# Autodesk Inventor assembly: EX_ONE
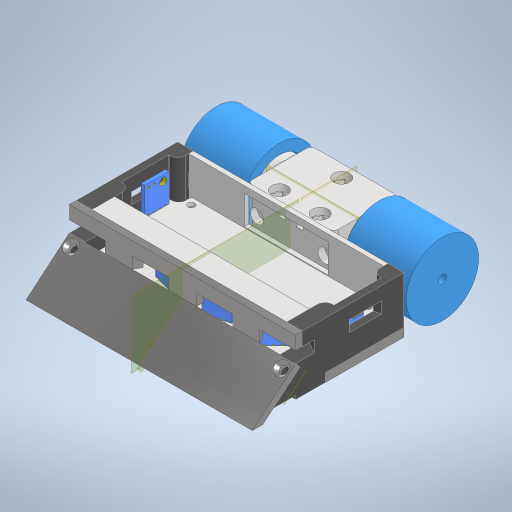
[picture p0: Inventor's stored thumbnail of the model, 512x512]
Saved by Autodesk Inventor 2023 (Build 270158000, 158)
## iProperties
Created: 2025-01-11
Part Number: EX_ONE
Document SubType Name: Assembly
Designer: kamil
Author: kamil
## Documents named in this file (15)
- C:\Users\kamil\Documents\PROJECTS - repos\EX_ONE_minisumo\mechanics\inventor_parts\EX_ONE.iam
- C:\Users\kamil\Documents\PROJECTS - repos\EX_ONE_minisumo\mechanics\inventor_parts\faulhaber_motor.ipt
- C:\Users\kamil\Documents\PROJECTS - repos\EX_ONE_minisumo\mechanics\inventor_parts\motors_mount.ipt
- C:\Users\kamil\Documents\PROJECTS - repos\EX_ONE_minisumo\mechanics\inventor_parts\kolo_tetsowe.ipt
- C:\Users\kamil\Documents\PROJECTS - repos\EX_ONE_minisumo\mechanics\inventor_parts\podstawa.ipt
- C:\Users\kamil\Documents\PROJECTS - repos\EX_ONE_minisumo\mechanics\inventor_parts\nóź.ipt
- C:\Users\kamil\Documents\PROJECTS - repos\EX_ONE_minisumo\mechanics\inventor_parts\TOF_VL53L0X (1).ipt
- C:\Users\kamil\Documents\PROJECTS - repos\EX_ONE_minisumo\mechanics\inventor_parts\pcb_pre.ipt
- C:\Users\kamil\Documents\PROJECTS - repos\EX_ONE_minisumo\mechanics\inventor_parts\minisunmo_testowe.ipt
- C:\Users\kamil\Documents\PROJECTS - repos\EX_ONE_minisumo\mechanics\inventor_parts\ściana.ipt
- C:\Users\kamil\Documents\PROJECTS - repos\EX_ONE_minisumo\mechanics\inventor_parts\ściana_MIR.ipt
- C:\Users\kamil\Documents\PROJECTS - repos\EX_ONE_minisumo\mechanics\inventor_parts\przod.ipt
- C:\Users\kamil\Documents\PROJECTS - repos\EX_ONE_minisumo\mechanics\inventor_parts\oslona.ipt
- C:\Users\kamil\Documents\PROJECTS - repos\EX_ONE_minisumo\mechanics\inventor_parts\pokrywa.ipt
- C:\Users\kamil\Documents\PROJECTS - repos\EX_ONE_minisumo\mechanics\inventor_parts\belka.ipt
## Components (21 placed, 14 different names)
1. faulhaber_motor:1 — Równoległe:31, Zestawiające:31
2. faulhaber_motor:2 — Równoległe:32, Zestawiające:30
3. motors_mount:1 — Zestawiające:9, Równoległe:23, Zestawiające:29, Równoległe:31, Równoległe:32, Zestawiające:30, Zestawiające:31, Zestawiające:32, Zestawiające:33
4. kolo_tetsowe:1 — Zestawiające:33, Równoległe:33
5. nóź:1
6. kolo_tetsowe:2 — Zestawiające:9, Zestawiające:32, Równoległe:34
7. pcb_pre:1 — Zestawiające:11, Równoległe:18
8. TOF_VL53L0X (1):1 — Zestawiające:11, Równoległe:10, Równoległe:11, Równoległe:15, Równoległe:18
9. TOF_VL53L0X (1):2 — Równoległe:11, Równoległe:15
10. TOF_VL53L0X (1):3 — Równoległe:10, Równoległe:14, Kątowe:5, Równoległe:24, Zestawiające:21, Zestawiające:23, Równoległe:26, Kątowe:8
11. TOF_VL53L0X (1):5 — Równoległe:25, Zestawiające:24, Kątowe:7, Zestawiające:26
12. TOF_VL53L0X (1):6 — Równoległe:14, Kątowe:5, Równoległe:26, Zestawiające:25, Kątowe:8, Zestawiające:27
13. minisunmo_testowe:1
14. ściana:1 — Zestawiające:18, Równoległe:21, Zestawiające:19, Równoległe:22, Symetria:1, Zestawiające:28, Równoległe:27, Równoległe:28, Równoległe:29, Równoległe:30, Równoległe:33
15. ściana_MIR:1 — Symetria:1, Równoległe:34
16. przod:1 — Zestawiające:18, Równoległe:21, Zestawiające:19, Kątowe:6, Zestawiające:22, Zestawiające:23, Zestawiające:26, Zestawiające:27
17. oslona:1 — Równoległe:22
18. pokrywa:1 — Równoległe:23
19. TOF_VL53L0X (1):7 — Kątowe:6, Równoległe:24, Zestawiające:20, Zestawiające:22, Równoległe:25, Kątowe:7
20. belka:1 — Zestawiające:28, Równoległe:27, Równoległe:28
21. podstawa:1 — Zestawiające:29, Równoległe:29, Równoległe:30
## Relationships (42: Flush 19, Mate 18, Angle 4, Symmetry 1)
- Zestawiające:9 [Mate]: motors_mount:1 ↔ kolo_tetsowe:2
- Zestawiające:11 [Mate]: pcb_pre:1 ↔ TOF_VL53L0X (1):1
- Równoległe:10 [Flush]: TOF_VL53L0X (1):1 ↔ TOF_VL53L0X (1):3
- Równoległe:11 [Flush]: TOF_VL53L0X (1):1 ↔ TOF_VL53L0X (1):2
- Równoległe:14 [Flush]: TOF_VL53L0X (1):3 ↔ TOF_VL53L0X (1):6
- Równoległe:15 [Flush]: TOF_VL53L0X (1):1 ↔ TOF_VL53L0X (1):2
- Kątowe:5 [Angle] (30 deg): TOF_VL53L0X (1):3 ↔ TOF_VL53L0X (1):6
- Równoległe:18 [Flush] (2 mm): pcb_pre:1 ↔ TOF_VL53L0X (1):1
- Zestawiające:18 [Mate]: ściana:1 ↔ przod:1
- Równoległe:21 [Flush]: ściana:1 ↔ przod:1
- Zestawiające:19 [Mate]: ściana:1 ↔ przod:1
- Równoległe:22 [Flush]: ściana:1 ↔ oslona:1
- Równoległe:23 [Flush]: motors_mount:1 ↔ pokrywa:1
- Kątowe:6 [Angle] (-195 deg): przod:1 ↔ TOF_VL53L0X (1):7
- Równoległe:24 [Flush]: TOF_VL53L0X (1):3 ↔ TOF_VL53L0X (1):7
- Symetria:1 [Symmetry]: ściana:1 ↔ ściana_MIR:1
- Zestawiające:20 [Mate] (10 mm): TOF_VL53L0X (1):7
- Zestawiające:21 [Mate] (-10 mm): TOF_VL53L0X (1):3
- Zestawiające:22 [Mate] (2 mm): przod:1 ↔ TOF_VL53L0X (1):7
- Zestawiające:23 [Mate] (2 mm): TOF_VL53L0X (1):3 ↔ przod:1
- Równoległe:25 [Flush]: TOF_VL53L0X (1):5 ↔ TOF_VL53L0X (1):7
- Równoległe:26 [Flush]: TOF_VL53L0X (1):3 ↔ TOF_VL53L0X (1):6
- Zestawiające:24 [Mate] (34 mm): TOF_VL53L0X (1):5
- Zestawiające:25 [Mate] (-34 mm): TOF_VL53L0X (1):6
- Kątowe:7 [Angle] (30 deg): TOF_VL53L0X (1):5 ↔ TOF_VL53L0X (1):7
- Kątowe:8 [Angle] (30 deg): TOF_VL53L0X (1):3 ↔ TOF_VL53L0X (1):6
- Zestawiające:26 [Mate] (5 mm): TOF_VL53L0X (1):5 ↔ przod:1
- Zestawiające:27 [Mate] (5 mm): TOF_VL53L0X (1):6 ↔ przod:1
- Zestawiające:28 [Mate]: ściana:1 ↔ belka:1
- Równoległe:27 [Flush]: ściana:1 ↔ belka:1
- Równoległe:28 [Flush]: ściana:1 ↔ belka:1
- Zestawiające:29 [Mate]: motors_mount:1 ↔ podstawa:1
- Równoległe:29 [Flush]: ściana:1 ↔ podstawa:1
- Równoległe:30 [Flush]: ściana:1 ↔ podstawa:1
- Równoległe:31 [Flush]: faulhaber_motor:1 ↔ motors_mount:1
- Równoległe:32 [Flush]: faulhaber_motor:2 ↔ motors_mount:1
- Zestawiające:30 [Mate]: faulhaber_motor:2 ↔ motors_mount:1
- Zestawiające:31 [Mate]: faulhaber_motor:1 ↔ motors_mount:1
- Zestawiające:32 [Mate]: motors_mount:1 ↔ kolo_tetsowe:2
- Zestawiające:33 [Mate]: motors_mount:1 ↔ kolo_tetsowe:1
- Równoległe:33 [Flush]: kolo_tetsowe:1 ↔ ściana:1
- Równoległe:34 [Flush]: kolo_tetsowe:2 ↔ ściana_MIR:1
